# Autodesk Inventor assembly: Assembly_Opentrons_Autofocus_Measure_v0
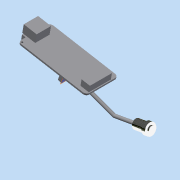
[picture p0: Inventor's stored thumbnail of the model, 180x180]
Saved by Autodesk Inventor 2019.4 (Build 234330000, 330)
## iProperties
Created: 2020-11-30
Part Number: Assembly_Opentrons_Autofocus_Measure_v0
Document SubType Name: Assembly
Designer: diederichbenedict
Author: diederichbenedict
## Documents named in this file (4)
- C:\Users\diederichbenedict\Dropbox\Dokumente\Promotion\PROJECTS\OPENTRONS\INVENTOR\Assembly_Opentrons_Autofocus_Measure_v0.iam
- C:\Users\diederichbenedict\Dropbox\Dokumente\Promotion\PROJECTS\OPENTRONS\INVENTOR\00_IR_Laserdiode.ipt
- C:\Users\diederichbenedict\Dropbox\Dokumente\Promotion\PROJECTS\OPENTRONS\INVENTOR\00_ESP32_CAM.ipt
- C:\Users\diederichbenedict\Dropbox\Dokumente\Promotion\PROJECTS\OPENTRONS\INVENTOR\00_Beampath_Autofocus.ipt
## Components (3 placed, 3 different names)
1. 00_ESP32_CAM:1 — Insert:1, Angle:1
2. 00_IR_Laserdiode:1 — Insert:2
3. 00_Beampath_Autofocus:1 — Insert:1, Angle:1, Insert:2
## Relationships (3: Insert 2, Angle 1)
- Insert:1: 00_ESP32_CAM:1 ↔ 00_Beampath_Autofocus:1
- Angle:1 (0 deg): 00_ESP32_CAM:1 ↔ 00_Beampath_Autofocus:1
- Insert:2: 00_IR_Laserdiode:1 ↔ 00_Beampath_Autofocus:1
